# Autodesk Inventor assembly: Closing Mechanism Arm Side
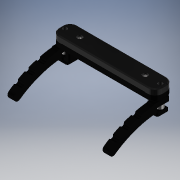
[picture p0: Inventor's stored thumbnail of the model, 180x180]
Saved by Autodesk Inventor 2019 (Build 230136000, 136)
## iProperties
Created: 2018-04-23
Part Number: Closing Mechanism Arm Side
Document SubType Name: Assembly
Designer: IEUser
Mass: 460.89 g
Surface Area: 638.171 cm^2
Volume: 151.871 cm^3
Density: 3.03475 g/cm^3
Author: IEUser
## Documents named in this file (13)
- C:\Users\IEUser\Desktop\Closing Mechanism\Closing Mechanism Arm Side.iam
- C:\Users\IEUser\Desktop\Closing Mechanism\Hard Plate.ipt
- C:\Users\IEUser\Desktop\Closing Mechanism\Stock Components\Automotion Components\P1207.030-014.ipt
- C:\Users\IEUser\Desktop\Closing Mechanism\Arm Simplified.ipt
- C:\Users\IEUser\Desktop\Closing Mechanism\Stock Components\Accu Group\SSCF-M8-22-A4.ipt
- C:\Users\IEUser\Desktop\Closing Mechanism\Rail.ipt
- C:\Users\IEUser\Desktop\Closing Mechanism\Stock Components\Accu Group\SSCF-M5-16-A4.ipt
- C:\Users\IEUser\Desktop\Closing Mechanism\Large Clamp.ipt
- C:\Users\IEUser\Desktop\Closing Mechanism\Small Clamp.ipt
- C:\Users\IEUser\Desktop\Closing Mechanism\Stock Components\Accu Group\SSK-M5-12-A4.ipt
- C:\Users\IEUser\Desktop\Closing Mechanism\Stock Components\Accu Group\SSK-M5-18-A4.ipt
- C:\Users\IEUser\Desktop\Closing Mechanism\Top Cover.ipt
- C:\Users\IEUser\Desktop\Closing Mechanism\Stock Components\Accu Group\SSCF-M5-10-A4.ipt
## Components (28 placed, 12 different names)
1. Hard Plate:1 — Mate:1, Mate:2, Mate:3, Mate:4, Tangent:1, Tangent:2, Tangent:3, Tangent:4, Mate:5, Mate:8, Mate:11, Mate:12, Mate:13, Mate:14, Mate:15, Mate:16, Insert:3, Insert:4, Insert:5, Insert:6, Mate:17, Mate:18, Mate:19, Mate:20, Mate:21, Mate:22, Mate:23, Mate:24, Mate:25
2. P1207.030-014:1 — Mate:1, Tangent:1, Mate:7
3. P1207.030-014:2 — Mate:2, Tangent:2, Mate:6
4. P1207.030-014:3 — Mate:3, Tangent:3, Mate:10
5. P1207.030-014:4 — Mate:4, Tangent:4, Mate:9
6. Arm Simplified:1 — Mate:5, Mate:6, Mate:7, Insert:1
7. Arm Simplified:2 — Mate:8, Mate:9, Mate:10, Insert:2
8. SSCF-M8-22-A4:1 — Insert:1
9. SSCF-M8-22-A4:2 — Insert:2
10. Rail:1 — Mate:11, Mate:12, Mate:13
11. Rail:2 — Mate:14, Mate:15, Mate:16
12. SSCF-M5-16-A4:1 — Insert:3
13. SSCF-M5-16-A4:2 — Insert:4
14. SSCF-M5-16-A4:3 — Insert:5
15. SSCF-M5-16-A4:4 — Insert:6
16. Large Clamp:1 — Mate:17, Mate:18, Mate:19, Insert:10, Insert:11, Insert:12, Insert:13, Insert:14
17. Small Clamp:1 — Mate:20, Mate:21, Mate:22, Insert:7, Insert:8, Insert:9
18. SSK-M5-12-A4:1 — Insert:7
19. SSK-M5-12-A4:2 — Insert:8
20. SSK-M5-12-A4:3 — Insert:9
21. SSK-M5-18-A4:1 — Insert:10
22. SSK-M5-18-A4:2 — Insert:11
23. SSK-M5-18-A4:3 — Insert:12
24. SSK-M5-18-A4:4 — Insert:13
25. SSK-M5-18-A4:5 — Insert:14
26. Top Cover:1 — Mate:23, Mate:24, Mate:25, Insert:15, Insert:16
27. SSCF-M5-10-A4:1 — Insert:15
28. SSCF-M5-10-A4:2 — Insert:16
## Relationships (45: Mate 25, Insert 16, Tangent 4)
- Mate:1: Hard Plate:1 ↔ P1207.030-014:1
- Mate:2: Hard Plate:1 ↔ P1207.030-014:2
- Mate:3: Hard Plate:1 ↔ P1207.030-014:3
- Mate:4: Hard Plate:1 ↔ P1207.030-014:4
- Tangent:1: Hard Plate:1 ↔ P1207.030-014:1
- Tangent:2: Hard Plate:1 ↔ P1207.030-014:2
- Tangent:3: Hard Plate:1 ↔ P1207.030-014:3
- Tangent:4: Hard Plate:1 ↔ P1207.030-014:4
- Mate:5: Hard Plate:1 ↔ Arm Simplified:1
- Mate:6: P1207.030-014:2 ↔ Arm Simplified:1
- Mate:7: P1207.030-014:1 ↔ Arm Simplified:1
- Mate:8: Hard Plate:1 ↔ Arm Simplified:2
- Mate:9: P1207.030-014:4 ↔ Arm Simplified:2
- Mate:10: P1207.030-014:3 ↔ Arm Simplified:2
- Insert:1: Arm Simplified:1 ↔ SSCF-M8-22-A4:1
- Insert:2: Arm Simplified:2 ↔ SSCF-M8-22-A4:2
- Mate:11: Hard Plate:1 ↔ Rail:1
- Mate:12: Hard Plate:1 ↔ Rail:1
- Mate:13: Hard Plate:1 ↔ Rail:1
- Mate:14: Hard Plate:1 ↔ Rail:2
- Mate:15: Hard Plate:1 ↔ Rail:2
- Mate:16: Hard Plate:1 ↔ Rail:2
- Insert:3: Hard Plate:1 ↔ SSCF-M5-16-A4:1
- Insert:4: Hard Plate:1 ↔ SSCF-M5-16-A4:2
- Insert:5: Hard Plate:1 ↔ SSCF-M5-16-A4:3
- Insert:6: Hard Plate:1 ↔ SSCF-M5-16-A4:4
- Mate:17: Hard Plate:1 ↔ Large Clamp:1
- Mate:18: Hard Plate:1 ↔ Large Clamp:1
- Mate:19: Hard Plate:1 ↔ Large Clamp:1
- Mate:20: Hard Plate:1 ↔ Small Clamp:1
- Mate:21: Hard Plate:1 ↔ Small Clamp:1
- Mate:22: Hard Plate:1 ↔ Small Clamp:1
- Insert:7: Small Clamp:1 ↔ SSK-M5-12-A4:1
- Insert:8: Small Clamp:1 ↔ SSK-M5-12-A4:2
- Insert:9: Small Clamp:1 ↔ SSK-M5-12-A4:3
- Insert:10: Large Clamp:1 ↔ SSK-M5-18-A4:1
- Insert:11: Large Clamp:1 ↔ SSK-M5-18-A4:2
- Insert:12: Large Clamp:1 ↔ SSK-M5-18-A4:3
- Insert:13: Large Clamp:1 ↔ SSK-M5-18-A4:4
- Insert:14: Large Clamp:1 ↔ SSK-M5-18-A4:5
- Mate:23: Hard Plate:1 ↔ Top Cover:1
- Mate:24: Hard Plate:1 ↔ Top Cover:1
- Mate:25: Hard Plate:1 ↔ Top Cover:1
- Insert:15: Top Cover:1 ↔ SSCF-M5-10-A4:1
- Insert:16: Top Cover:1 ↔ SSCF-M5-10-A4:2
